# Autodesk Inventor assembly: Рама_02
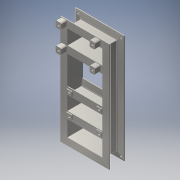
[picture p0: Inventor's stored thumbnail of the model, 180x180]
Saved by Autodesk Inventor 2016 (Build 200138000, 138)
## iProperties
Created: 2021-05-08
Part Number: Рама_02
Material: Типовые
Document SubType Name: Assembly
Designer: Лол
Mass: 21309.1 g
Surface Area: 9446.14 cm^2
Volume: 2866.96 cm^3
Density: 7.43264 g/cm^3
_SolveAssemblyDoc: Frame Generator Solve Assembly
_Version: 15.0.0
Author: Лол
## Documents named in this file (5)
- C:\Users\Лол\Documents\Inventor\course_work\Рама_02.iam
- C:\Users\Лол\Documents\Inventor\course_work\рама_01.ipt
- C:\Users\Лол\Documents\Inventor\course_work\Рама_02\Frame\Frame0001.iam
- C:\Users\Лол\Documents\Inventor\course_work\платик под редуктор.ipt
- C:\Users\Лол\Documents\Inventor\course_work\платик под двигатель.ipt
## Components (10 placed, 4 different names)
1. рама_01:1
2. Frame0001:1 [sub-assembly] — Совмещение:1, Совмещение:2, Совмещение:3, Совмещение:4, Угол:1, Угол:2, Совмещение:5, Совмещение:6, Совмещение:7, Совмещение:8, Угол:3, Угол:4, Совмещение:9, Совмещение:10, Совмещение:11, Совмещение:12, Совмещение:13, Совмещение:14, Совмещение:15, Совмещение:16, Угол:5, Угол:6, Угол:7, Угол:8, Заподлицо:1
3. платик под редуктор:1 — Совмещение:3, Совмещение:4, Угол:1
4. платик под редуктор:2 — Совмещение:1, Совмещение:2, Угол:2
5. платик под редуктор:3 — Совмещение:6, Совмещение:7, Угол:4
6. платик под редуктор:4 — Совмещение:5, Совмещение:8, Угол:3
7. платик под двигатель:1 — Совмещение:9, Совмещение:15, Угол:7
8. платик под двигатель:2 — Совмещение:11, Совмещение:13, Угол:6
9. платик под двигатель:3 — Совмещение:10, Совмещение:16, Угол:8
10. платик под двигатель:4 — Совмещение:12, Совмещение:14, Угол:5
## Relationships (25: Mate 16, Angle 8, Flush 1)
- Совмещение:1 [Mate]: Frame0001:1 ↔ платик под редуктор:2
- Совмещение:2 [Mate]: Frame0001:1 ↔ платик под редуктор:2
- Совмещение:3 [Mate]: Frame0001:1 ↔ платик под редуктор:1
- Совмещение:4 [Mate]: Frame0001:1 ↔ платик под редуктор:1
- Угол:1 [Angle] (90 deg): Frame0001:1 ↔ платик под редуктор:1
- Угол:2 [Angle] (180 deg): Frame0001:1 ↔ платик под редуктор:2
- Совмещение:5 [Mate]: Frame0001:1 ↔ платик под редуктор:4
- Совмещение:6 [Mate]: Frame0001:1 ↔ платик под редуктор:3
- Совмещение:7 [Mate]: Frame0001:1 ↔ платик под редуктор:3
- Совмещение:8 [Mate]: Frame0001:1 ↔ платик под редуктор:4
- Угол:3 [Angle] (0 deg): Frame0001:1 ↔ платик под редуктор:4
- Угол:4 [Angle] (180 deg): Frame0001:1 ↔ платик под редуктор:3
- Совмещение:9 [Mate]: Frame0001:1 ↔ платик под двигатель:1
- Совмещение:10 [Mate]: Frame0001:1 ↔ платик под двигатель:3
- Совмещение:11 [Mate]: Frame0001:1 ↔ платик под двигатель:2
- Совмещение:12 [Mate]: Frame0001:1 ↔ платик под двигатель:4
- Совмещение:13 [Mate]: Frame0001:1 ↔ платик под двигатель:2
- Совмещение:14 [Mate]: Frame0001:1 ↔ платик под двигатель:4
- Совмещение:15 [Mate]: Frame0001:1 ↔ платик под двигатель:1
- Совмещение:16 [Mate]: Frame0001:1 ↔ платик под двигатель:3
- Угол:5 [Angle] (0 deg): Frame0001:1 ↔ платик под двигатель:4
- Угол:6 [Angle] (0 deg): Frame0001:1 ↔ платик под двигатель:2
- Угол:7 [Angle] (0 deg): Frame0001:1 ↔ платик под двигатель:1
- Угол:8 [Angle] (0 deg): Frame0001:1 ↔ платик под двигатель:3
- Заподлицо:1 [Flush] (-85 mm): Frame0001:1
